# Autodesk Inventor assembly: Main_Top
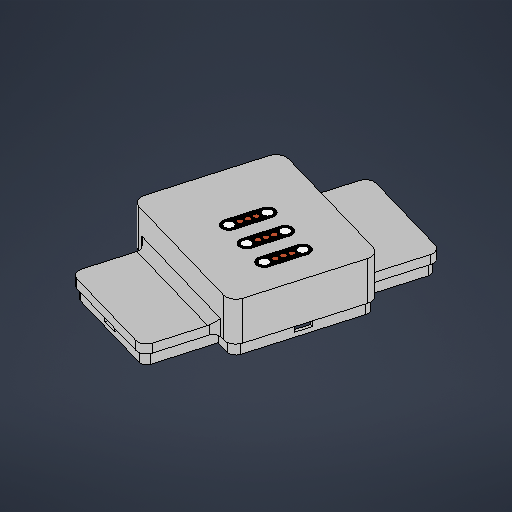
[picture p0: Inventor's stored thumbnail of the model, 512x512]
Saved by Autodesk Inventor 2026 (Build 300175000, 175)
## iProperties
Created: 2025-04-14
Part Number: Main_Top
Document SubType Name: Assembly
Designer: ct_vi
Author: ct_vi
## Documents named in this file (4)
- C:\Users\ct_vi\Documents\Capstone_Research_3D_Files\Main_Top.iam
- C:\Users\ct_vi\Documents\Capstone_Research_3D_Files\Body_Up.ipt
- C:\Users\ct_vi\Documents\Capstone_Research_3D_Files\Pogo_Set1.iam
- C:\Users\ct_vi\Documents\Capstone_Research_3D_Files\6x3_Magnet.ipt
## Components (6 placed, 3 different names)
1. Body_Up:1 — Mate:1, Flush:1, Flush:2, Flush:3, Insert:1, Insert:2, Insert:3, Mate:2, Mate:3, Mate:4, Mate:5
2. Pogo_Set1:1 [sub-assembly] — Flush:3, Insert:3, Mate:2
3. Pogo_Set1:2 [sub-assembly] — Mate:1, Flush:1, Mate:3
4. Pogo_Set1:3 [sub-assembly] — Flush:2, Mate:4, Mate:5
5. 6x3_Magnet:1 — Insert:1
6. 6x3_Magnet:2 — Insert:2
## Relationships (11: Mate 5, Flush 3, Insert 3)
- Mate:1: Body_Up:1 ↔ Pogo_Set1:2
- Flush:1: Body_Up:1 ↔ Pogo_Set1:2
- Flush:2: Body_Up:1 ↔ Pogo_Set1:3
- Flush:3: Body_Up:1 ↔ Pogo_Set1:1
- Insert:1: Body_Up:1 ↔ 6x3_Magnet:1
- Insert:2: Body_Up:1 ↔ 6x3_Magnet:2
- Insert:3: Body_Up:1 ↔ Pogo_Set1:1
- Mate:2: Body_Up:1 ↔ Pogo_Set1:1
- Mate:3: Body_Up:1 ↔ Pogo_Set1:2
- Mate:4: Body_Up:1 ↔ Pogo_Set1:3
- Mate:5: Body_Up:1 ↔ Pogo_Set1:3
